# Autodesk Inventor assembly: Conjunto Caja-Vaso-TapaVaso
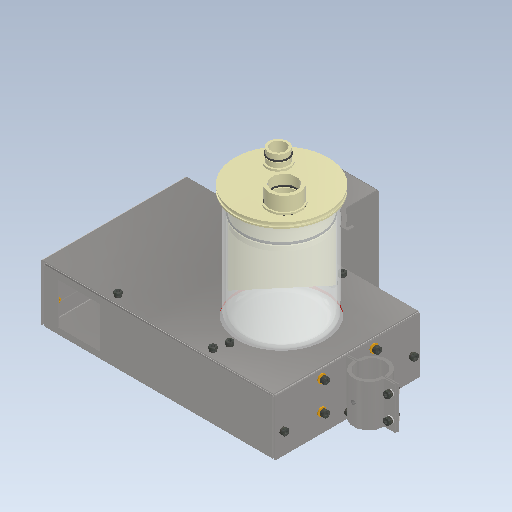
[picture p0: Inventor's stored thumbnail of the model, 512x512]
Saved by Autodesk Inventor 2020.3 (Build 243373000, 373)
## iProperties
Created: 2020-07-13
Part Number: Conjunto Caja-Vaso-TapaVaso
Document SubType Name: Assembly
Designer: Bruno
Author: Bruno
## Documents named in this file (4)
- C:\Users\Bruno\Desktop\CNAF\CNAF-3\Conjunto Caja-Vaso-TapaVaso.iam
- C:\Users\Bruno\Desktop\CNAF\CNAF-3\Conjuntoi Caja CNAF.iam
- C:\Users\Bruno\Desktop\CNAF\CNAF-3\Vaso precipitado 600ml-De90-Di84-H120.ipt
- C:\Users\Bruno\Desktop\CNAF\CNAF-3\Conjunto Tapa Vaso.iam
## Components (3 placed, 3 different names)
1. Conjuntoi Caja CNAF:1 [sub-assembly] — Cylindrical:1
2. Vaso precipitado 600ml-De90-Di84-H120:1 — Cylindrical:1, Cylindrical:2
3. Conjunto Tapa Vaso:1 [sub-assembly] — Cylindrical:2
## Relationships (2: CylindricalJoint 2)
- Cylindrical:1: Conjuntoi Caja CNAF:1 ↔ Vaso precipitado 600ml-De90-Di84-H120:1
- Cylindrical:2: Vaso precipitado 600ml-De90-Di84-H120:1 ↔ Conjunto Tapa Vaso:1
